# Autodesk Inventor assembly: MotorEncoderAssembly
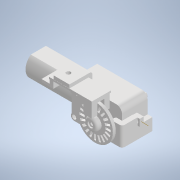
[picture p0: Inventor's stored thumbnail of the model, 180x180]
Saved by Autodesk Inventor 2022 (Build 260153070, 153G)
## iProperties
Created: 2021-11-27
Part Number: MotorEncoderAssembly
Document SubType Name: Assembly
Designer: a laptop
Author: a laptop
## Documents named in this file (8)
- C:\Users\a laptop\Desktop\SumoBot\sumobotENCODER\MotorEncoderAssembly.iam
- C:\Users\a laptop\Desktop\SumoBot\sumobotENCODER\REF_PART\LM393 encoder.ipt
- C:\Users\a laptop\Desktop\SumoBot\sumobotENCODER\REF_PART\TT encoder disk.ipt
- C:\Users\a laptop\Desktop\SumoBot\sumobotENCODER\REF_PART\TT motor output.ipt
- C:\Users\a laptop\Desktop\SumoBot\sumobotENCODER\MotorEncoderBracket.ipt
- C:\Users\a laptop\Desktop\SumoBot\sumobotENCODER\REF_PART\TTencoderspacer.ipt
- C:\Users\a laptop\Desktop\SumoBot\sumobotENCODER\REF_PART\TTencodercap.ipt
- C:\Users\a laptop\Desktop\SumoBot\sumobotENCODER\REF_PART\TTmotor.ipt
## Components (7 placed, 7 different names)
1. LM393 encoder:1 — Angle:2, Angle:3, Mate:3, Mate:8, Tangent:1
2. TT encoder disk:1 — Mate:1, Angle:1, Flush:1, Mate:2, Mate:3, Tangent:1
3. TT motor output:1 — Mate:1, Angle:1, Flush:1, Mate:2, Angle:2, Angle:3, Mate:4, Mate:5, Flush:2, Flush:3, Flush:4, Mate:10, Mate:11
4. MotorEncoderBracket:1 — Flush:2
5. TTencoderspacer:1 — Flush:3
6. TTencodercap:1 — Flush:4
7. TTmotor:1 — Mate:10, Mate:11
## Relationships (19: Mate 11, Flush 4, Angle 3, Tangent 1)
- Mate:1: TT encoder disk:1 ↔ TT motor output:1
- Angle:1 (0 deg): TT encoder disk:1 ↔ TT motor output:1
- Flush:1: TT encoder disk:1 ↔ TT motor output:1
- Mate:2: TT encoder disk:1 ↔ TT motor output:1
- Angle:2 (180 deg): LM393 encoder:1 ↔ TT motor output:1
- Angle:3 (180 deg): LM393 encoder:1 ↔ TT motor output:1
- Mate:3 (1.5 mm): LM393 encoder:1 ↔ TT encoder disk:1
- Mate:4: TT motor output:1
- Mate:5: TT motor output:1
- Mate:6
- Mate:7
- Mate:8: LM393 encoder:1
- Mate:9 (0.925 mm)
- Tangent:1 (1.5 mm): LM393 encoder:1 ↔ TT encoder disk:1
- Flush:2: TT motor output:1 ↔ MotorEncoderBracket:1
- Flush:3: TT motor output:1 ↔ TTencoderspacer:1
- Flush:4: TT motor output:1 ↔ TTencodercap:1
- Mate:10: TT motor output:1 ↔ TTmotor:1
- Mate:11: TT motor output:1 ↔ TTmotor:1
